# Autodesk Inventor assembly: Expansor
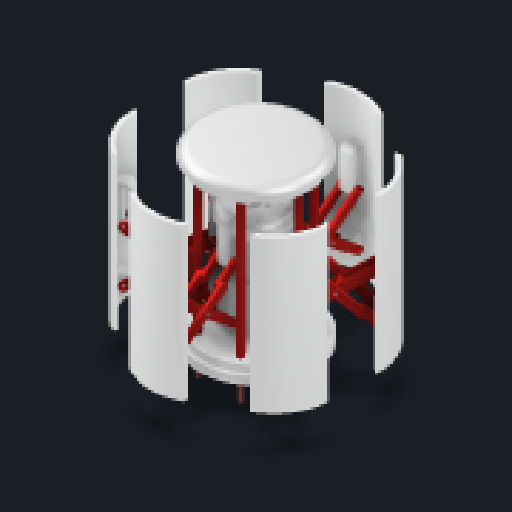
[picture p0: Inventor's stored thumbnail of the model, 512x512]
Saved by Autodesk Inventor 2025.3 (Build 293356030, 356C)
## iProperties
Created: 2024-12-25
Part Number: Expansor
Document SubType Name: Assembly
Designer: Usuario
Author: Usuario
## Documents named in this file (16)
- C:\Users\santa\OneDrive - Universidad de los Andes\Robocol\Flotador\V3\Expansor.iam
- C:\Users\santa\OneDrive - Universidad de los Andes\Robocol\Flotador\V3\Expansor\Clavija.ipt
- C:\Users\santa\OneDrive - Universidad de los Andes\Robocol\Flotador\V3\Expansor\Columnas.ipt
- C:\Users\santa\OneDrive - Universidad de los Andes\Robocol\Flotador\V3\Expansor\Corredera I.ipt
- C:\Users\santa\OneDrive - Universidad de los Andes\Robocol\Flotador\V3\Expansor\Corredera II.ipt
- C:\Users\santa\OneDrive - Universidad de los Andes\Robocol\Flotador\V3\Expansor\Corredor.ipt
- C:\Users\santa\OneDrive - Universidad de los Andes\Robocol\Flotador\V3\Expansor\Paletas.ipt
- C:\Users\santa\OneDrive - Universidad de los Andes\Robocol\Flotador\V3\Expansor\Soporte.ipt
- C:\Users\santa\OneDrive - Universidad de los Andes\Robocol\Flotador\V3\Expansor\Tapa.ipt
- C:\Users\santa\OneDrive - Universidad de los Andes\Robocol\Flotador\Downloads\screw nut 8mm\screw nut 8mm.ipt
- C:\Users\santa\OneDrive - Universidad de los Andes\Robocol\Flotador\V3\Expansor\AIP\FEA\exazi096o.fins
- C:\Users\santa\OneDrive - Universidad de los Andes\Robocol\Flotador\V3\Expansor\AIP\FEA\exazi096o.fsat
- C:\Users\santa\OneDrive - Universidad de los Andes\Robocol\Flotador\V3\Expansor\AIP\FEA\exazi096o.ftes
- C:\Users\santa\OneDrive - Universidad de los Andes\Robocol\Flotador\V3\Expansor\AIP\FEA\exazi096o.fwiz
- C:\Users\santa\OneDrive - Universidad de los Andes\Robocol\Flotador\V3\Expansor\AIP\FEA\exazi09pc.fmsh
- C:\Users\santa\OneDrive - Universidad de los Andes\Robocol\Flotador\V3\Expansor\AIP\FEA\exazi09pd.fres
## Components (34 placed, 9 different names)
1. Corredor:1 — ANIMAR, De rotación:5, Rígido:3
2. Soporte:1 — Nivelación:1, Coincidencia:1, Nivelación:2, Rígido:1, ANIMAR, De rotación:3, Coincidencia:2
3. Tapa:1 — De rotación:6
4. screw nut 8mm:1 — Rígido:3
5. Paletas:1 — De rotación:4, Coincidencia:2, Tangente:1
6. Corredera I:1 — De rotación:1, De rotación:4, De rotación:5
7. Corredera II:1 — Rígido:2, De rotación:1, De rotación:3, Tangente:1
8. Clavija:1 — Rígido:2
9. Columnas:1 — Rígido:1, De rotación:6
10. Paletas:2
11. Corredera I:2
12. Corredera II:2
13. Clavija:2
14. Columnas:2
15. Paletas:3
16. Corredera I:3
17. Corredera II:3
18. Clavija:3
19. Columnas:3
20. Paletas:4
21. Corredera I:4
22. Corredera II:4
23. Clavija:4
24. Columnas:4
25. Paletas:5
26. Corredera I:5
27. Corredera II:5
28. Clavija:5
29. Columnas:5
30. Paletas:6
31. Corredera I:6
32. Corredera II:6
33. Clavija:6
34. Columnas:6
## Component patterns: (6 elements, first: Paletas:1 + Corredera I:1 + Corredera II:1 + Clavija:1 + Columnas:1)
## Relationships (14: RevoluteJoint 5, WeldJoint 3, Flush 2, Mate 2, CylindricalJoint 1, Tangent 1)
- Nivelación:1 [Flush]: Soporte:1
- Coincidencia:1 [Mate]: Soporte:1
- Nivelación:2 [Flush]: Soporte:1
- Rígido:1 [WeldJoint]: Soporte:1 ↔ Columnas:1
- Rígido:2 [WeldJoint]: Corredera II:1 ↔ Clavija:1
- De rotación:1 [RevoluteJoint]: Corredera I:1 ↔ Corredera II:1
- ANIMAR [CylindricalJoint]: Corredor:1 ↔ Soporte:1
- De rotación:3 [RevoluteJoint]: Soporte:1 ↔ Corredera II:1
- De rotación:4 [RevoluteJoint]: Paletas:1 ↔ Corredera I:1
- Coincidencia:2 [Mate]: Soporte:1 ↔ Paletas:1
- Tangente:1: Paletas:1 ↔ Corredera II:1
- De rotación:5 [RevoluteJoint]: Corredor:1 ↔ Corredera I:1
- De rotación:6 [RevoluteJoint]: Tapa:1 ↔ Columnas:1
- Rígido:3 [WeldJoint]: Corredor:1 ↔ screw nut 8mm:1
